# Autodesk Inventor assembly: Electrical panel
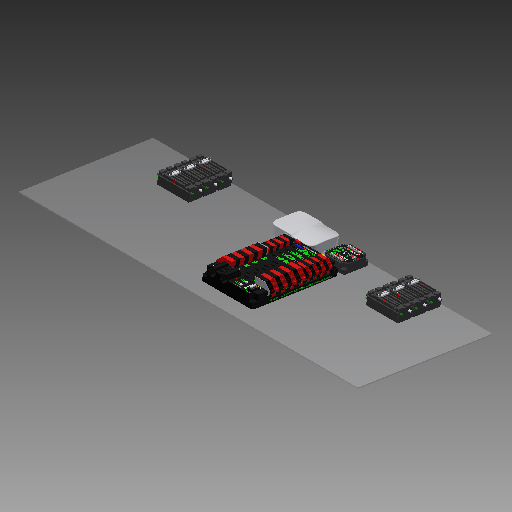
[picture p0: Inventor's stored thumbnail of the model, 512x512]
Saved by Autodesk Inventor 2019 (Build 230136000, 136)
## iProperties
Created: 2019-03-18
Part Number: Electrical panel
Document SubType Name: Assembly
Designer: josh
Mass: 1274.18 g
Surface Area: 9544.16 cm^2
Volume: 1274.18 cm^3
Density: 1 g/cm^3
Author: josh
## Documents named in this file (6)
- D:\Synthesis Robots\Epsilon\Chasis\Electrical panel.iam
- D:\Synthesis Robots\Epsilon\Chasis\Plexi Glass.ipt
- D:\Synthesis Robots\Epsilon\Chasis\OM5P-AN.ipt
- D:\Synthesis Robots\Epsilon\Chasis\Power_Distribution_Panel_217-4244 (1).ipt
- D:\Synthesis Robots\Epsilon\Chasis\Voltage_Regulator_Module_217-4245.ipt
- D:\Synthesis Robots\Epsilon\Chasis\Talons\Talon_SRX_217-8080_No_Wires.iam
## Components (10 placed, 5 different names)
1. Plexi Glass:1
2. OM5P-AN:1
3. Power_Distribution_Panel_217-4244 (1):1
4. Voltage_Regulator_Module_217-4245:1
5. Talon_SRX_217-8080_No_Wires:1 [sub-assembly]
6. Talon_SRX_217-8080_No_Wires:2 [sub-assembly]
7. Talon_SRX_217-8080_No_Wires:3 [sub-assembly]
8. Talon_SRX_217-8080_No_Wires:4 [sub-assembly]
9. Talon_SRX_217-8080_No_Wires:5 [sub-assembly]
10. Talon_SRX_217-8080_No_Wires:6 [sub-assembly]
## Relationships (24: Mate 12, Tangent 6, Flush 6)
- [Mate]: Plexi Glass:1 ↔ OM5P-AN:1
- [Tangent] (6.35 mm): Plexi Glass:1 ↔ OM5P-AN:1
- [Tangent] (6.35 mm): Plexi Glass:1 ↔ OM5P-AN:1
- [Mate]: Plexi Glass:1 ↔ Power_Distribution_Panel_217-4244 (1):1
- [Mate]: Plexi Glass:1 ↔ Voltage_Regulator_Module_217-4245:1
- [Mate]: Plexi Glass:1 ↔ Talon_SRX_217-8080_No_Wires:2
- [Mate]: Plexi Glass:1 ↔ Talon_SRX_217-8080_No_Wires:1
- [Mate]: Plexi Glass:1 ↔ Talon_SRX_217-8080_No_Wires:3
- [Flush]: Talon_SRX_217-8080_No_Wires:2 ↔ Talon_SRX_217-8080_No_Wires:3
- [Flush]: Talon_SRX_217-8080_No_Wires:1 ↔ Talon_SRX_217-8080_No_Wires:3
- [Tangent] (6.35 mm): Talon_SRX_217-8080_No_Wires:2 ↔ Talon_SRX_217-8080_No_Wires:3
- [Tangent] (6.35 mm): Talon_SRX_217-8080_No_Wires:1 ↔ Talon_SRX_217-8080_No_Wires:2
- [Mate] (-6.35 mm): Plexi Glass:1 ↔ Talon_SRX_217-8080_No_Wires:1
- [Mate] (-6.35 mm): Plexi Glass:1 ↔ Voltage_Regulator_Module_217-4245:1
- [Flush]: Talon_SRX_217-8080_No_Wires:5 ↔ Talon_SRX_217-8080_No_Wires:6
- [Flush]: Talon_SRX_217-8080_No_Wires:4 ↔ Talon_SRX_217-8080_No_Wires:6
- [Tangent] (6.35 mm): Talon_SRX_217-8080_No_Wires:5 ↔ Talon_SRX_217-8080_No_Wires:6
- [Tangent] (6.35 mm): Talon_SRX_217-8080_No_Wires:4 ↔ Talon_SRX_217-8080_No_Wires:5
- [Flush]: Talon_SRX_217-8080_No_Wires:4 ↔ Talon_SRX_217-8080_No_Wires:6
- [Flush]: Talon_SRX_217-8080_No_Wires:4 ↔ Talon_SRX_217-8080_No_Wires:5
- [Mate]: Plexi Glass:1 ↔ Talon_SRX_217-8080_No_Wires:4
- [Mate]: Plexi Glass:1 ↔ Talon_SRX_217-8080_No_Wires:5
- [Mate]: Plexi Glass:1 ↔ Talon_SRX_217-8080_No_Wires:6
- [Mate] (-6.35 mm): Plexi Glass:1 ↔ Talon_SRX_217-8080_No_Wires:4
## Named parameters: d886_d878 = 0 mm, d887_d879 = 0 mm, d888_d880 = 6.35 mm, d889_d881 = 6.35 mm
